# Autodesk Inventor assembly: CameraUnit
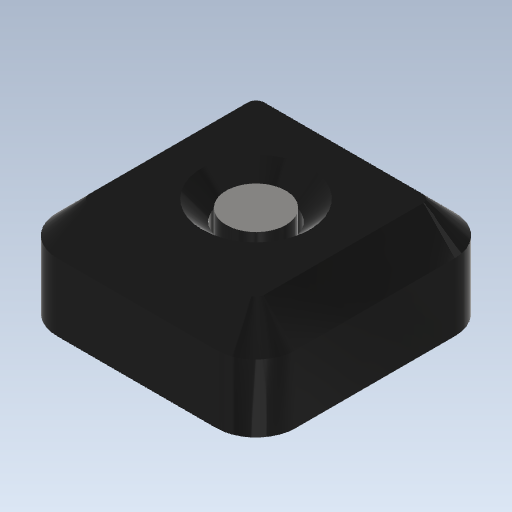
[picture p0: Inventor's stored thumbnail of the model, 512x512]
Saved by Autodesk Inventor 2020.4 (Build 244396000, 396)
## iProperties
Created: 2021-12-31
Part Number: CameraUnit
Document SubType Name: Assembly
Designer: Masato Kubotera
Mass: 44.5001 g
Surface Area: 252.134 cm^2
Volume: 70.4636 cm^3
Density: 0.631533 g/cm^3
Author: Masato Kubotera
## Documents named in this file (7)
- C:\Users\Masato\Documents\Inventor\CIT Brains_Inventor\OpenPlatform_ver3_0 - ve4_1 branch\UpperBody\Head\CameraUnit.iam
- C:\Users\Masato\Documents\Inventor\CIT Brains_Inventor\OpenPlatform_ver3_0 - ve4_1 branch\UpperBody\Head\Camera_root_frame_.ipt
- C:\Users\Masato\Documents\Inventor\CIT Brains_Inventor\OpenPlatform_ver3_0 - ve4_1 branch\Ready_Made\InsertNut\BRM2-4.1.ipt
- C:\Users\Masato\Documents\Inventor\CIT Brains_Inventor\OpenPlatform_ver3_0 - ve4_1 branch\Ready_Made\KBCR-S08MM.ipt
- C:\Users\Masato\Documents\Inventor\CIT Brains_Inventor\OpenPlatform_ver3_0 - ve4_1 branch\Ready_Made\Screw\M2-6.ipt
- C:\Users\Masato\Documents\Inventor\CIT Brains_Inventor\OpenPlatform_ver3_0 - ve4_1 branch\UpperBody\Head\Camera_cover_.ipt
- C:\Users\Masato\Documents\Inventor\CIT Brains_Inventor\OpenPlatform_ver3_0 - ve4_1 branch\Ready_Made\InsertNut\UD-43040.ipt
## Components (15 placed, 6 different names)
1. Camera_root_frame_:1 — 挿入:1, 挿入:2, 挿入:3, 挿入:4, 挿入:17, 挿入:18, 挿入:19, 挿入:20
2. BRM2-4.1:1 — 挿入:1, 挿入:5
3. BRM2-4.1:2 — 挿入:2, 挿入:6
4. BRM2-4.1:3 — 挿入:3, 挿入:7
5. BRM2-4.1:4 — 挿入:4, 挿入:8
6. KBCR-S08MM:1 — 挿入:5, 挿入:6, 挿入:7, 挿入:8, 挿入:9, 挿入:10, 挿入:11, 挿入:12
7. M2-6:1 — 挿入:9
8. M2-6:2 — 挿入:10
9. M2-6:3 — 挿入:11
10. M2-6:4 — 挿入:12
11. Camera_cover_:1 — 挿入:13, 挿入:14, 挿入:15, 挿入:16
12. UD-43040:1 — 挿入:13, 挿入:18
13. UD-43040:2 — 挿入:14, 挿入:17
14. UD-43040:3 — 挿入:15, 挿入:20
15. UD-43040:4 — 挿入:16, 挿入:19
## Relationships (20: Insert 20)
- 挿入:1 [Insert]: Camera_root_frame_:1 ↔ BRM2-4.1:1
- 挿入:2 [Insert]: Camera_root_frame_:1 ↔ BRM2-4.1:2
- 挿入:3 [Insert]: Camera_root_frame_:1 ↔ BRM2-4.1:3
- 挿入:4 [Insert]: Camera_root_frame_:1 ↔ BRM2-4.1:4
- 挿入:5 [Insert]: BRM2-4.1:1 ↔ KBCR-S08MM:1
- 挿入:6 [Insert]: BRM2-4.1:2 ↔ KBCR-S08MM:1
- 挿入:7 [Insert]: BRM2-4.1:3 ↔ KBCR-S08MM:1
- 挿入:8 [Insert]: BRM2-4.1:4 ↔ KBCR-S08MM:1
- 挿入:9 [Insert]: KBCR-S08MM:1 ↔ M2-6:1
- 挿入:10 [Insert]: KBCR-S08MM:1 ↔ M2-6:2
- 挿入:11 [Insert]: KBCR-S08MM:1 ↔ M2-6:3
- 挿入:12 [Insert]: KBCR-S08MM:1 ↔ M2-6:4
- 挿入:13 [Insert]: Camera_cover_:1 ↔ UD-43040:1
- 挿入:14 [Insert]: Camera_cover_:1 ↔ UD-43040:2
- 挿入:15 [Insert]: Camera_cover_:1 ↔ UD-43040:3
- 挿入:16 [Insert]: Camera_cover_:1 ↔ UD-43040:4
- 挿入:17 [Insert]: Camera_root_frame_:1 ↔ UD-43040:2
- 挿入:18 [Insert]: Camera_root_frame_:1 ↔ UD-43040:1
- 挿入:19 [Insert]: Camera_root_frame_:1 ↔ UD-43040:4
- 挿入:20 [Insert]: Camera_root_frame_:1 ↔ UD-43040:3
